# Autodesk Inventor assembly: WheelAssembly
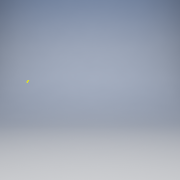
[picture p0: Inventor's stored thumbnail of the model, 180x180]
Saved by Autodesk Inventor 2016 (Build 200138000, 138)
## iProperties
Created: 2016-09-10
Part Number: WheelAssembly
Document SubType Name: Assembly
Designer: RoboticsUser
Author: RoboticsUser
## Documents named in this file (11)
- C:\Robotics\2016-17_CAD\WheelAssembly.iam
- C:\Robotics\CAD\2015-16\custom cad parts\am-2648_4inWheel8mmHub.ipt
- C:\Robotics\CAD\2015-16\COTSParts\Actobotics\545 parts\545556.ipt
- C:\Robotics\CAD\2015-16\COTSParts\Actobotics\615 parts\615102.ipt
- C:\Robotics\CAD\2015-16\COTSParts\Actobotics\634 parts\634080.ipt
- C:\Users\RoboticsUser\Desktop\2015-16 CAD\COTSParts\Actobotics\am-2964NeveRest.ipt
- C:\Users\RoboticsUser\Desktop\2015-16 CAD\COTSParts\Actobotics\615 parts\615114.ipt
- C:\Users\RoboticsUser\Desktop\2015-16 CAD\COTSParts\Tetrix\tetrix-motor-mounts-1.snapshot.1\Tetrex 2pc motor mount.ipt
- C:\Robotics\2016-17_CAD\DriveTrainPlate.iam
- C:\Robotics\CAD\2015-16\COTSParts\Actobotics\545 parts\545456.ipt
- C:\Robotics\CAD\2015-16\COTSParts\Bosch Extrusion\Bosch 20x20.ipt
## Components (26 placed, 10 different names)
1. am-2648_4inWheel8mmHub:2 — Insert:45, Insert:49
2. 545556:2 — Insert:48, Insert:51
3. 634080:1
4. 615102:3
5. 615102:4 — Insert:44
6. 634080:2 — Insert:41, Insert:47
7. am-2648_4inWheel8mmHub:3 — Insert:56, Insert:57
8. 545556:6 — Insert:52, Insert:55
9. 615102:5 — Insert:54, Insert:57
10. 634080:3 — Insert:40, Insert:46
11. am-2964NeveRest:2 — Insert:27, Insert:60
12. 545556:8 — Insert:61
13. 615114:2 — Insert:60, Insert:61
14. 615114:3 — Insert:58, Insert:59
15. 545556:9 — Insert:59
16. am-2964NeveRest:3 — Insert:28, Insert:58
17. Tetrex 2pc motor mount:1 — Insert:27, Insert:31, Insert:32, Insert:33
18. Tetrex 2pc motor mount:2 — Insert:28, Insert:34, Insert:35
19. DriveTrainPlate:1 [sub-assembly] — Insert:31, Insert:32, Insert:33, Insert:34, Insert:35, Insert:46, Insert:47, Mate:1, Flush:1, Flush:2
20. DriveTrainPlate:2 [sub-assembly] — Insert:40, Insert:41, Insert:51, Insert:52
21. 545556:10 — Insert:44, Insert:45
22. 545456:1 — Insert:49, Insert:48
23. 545456:2
24. 545456:3 — Insert:55, Insert:56
25. 545556:11 — Insert:54
26. Bosch 20x20:1 — Mate:1, Flush:1, Flush:2
## Relationships (28: Insert 25, Flush 2, Mate 1)
- Insert:27: am-2964NeveRest:2 ↔ Tetrex 2pc motor mount:1
- Insert:28: am-2964NeveRest:3 ↔ Tetrex 2pc motor mount:2
- Insert:31: Tetrex 2pc motor mount:1 ↔ DriveTrainPlate:1
- Insert:32: Tetrex 2pc motor mount:1 ↔ DriveTrainPlate:1
- Insert:33: Tetrex 2pc motor mount:1 ↔ DriveTrainPlate:1
- Insert:34: Tetrex 2pc motor mount:2 ↔ DriveTrainPlate:1
- Insert:35: Tetrex 2pc motor mount:2 ↔ DriveTrainPlate:1
- Insert:40: 634080:3 ↔ DriveTrainPlate:2
- Insert:41: 634080:2 ↔ DriveTrainPlate:2
- Insert:44: 615102:4 ↔ 545556:10
- Insert:45 (9.525 mm): am-2648_4inWheel8mmHub:2 ↔ 545556:10
- Insert:46 (2.3368 mm): 634080:3 ↔ DriveTrainPlate:1
- Insert:47 (2.3368 mm): 634080:2 ↔ DriveTrainPlate:1
- Insert:48: 545556:2 ↔ 545456:1
- Insert:49: am-2648_4inWheel8mmHub:2 ↔ 545456:1
- Insert:51 (9.525 mm): 545556:2 ↔ DriveTrainPlate:2
- Insert:52 (9.525 mm): 545556:6 ↔ DriveTrainPlate:2
- Insert:54: 615102:5 ↔ 545556:11
- Insert:55: 545556:6 ↔ 545456:3
- Insert:56: am-2648_4inWheel8mmHub:3 ↔ 545456:3
- Insert:57 (9.525 mm): am-2648_4inWheel8mmHub:3 ↔ 615102:5
- Insert:58 (16.637 mm): 615114:3 ↔ am-2964NeveRest:3
- Insert:59: 615114:3 ↔ 545556:9
- Insert:60 (16.637 mm): am-2964NeveRest:2 ↔ 615114:2
- Insert:61: 545556:8 ↔ 615114:2
- Mate:1: DriveTrainPlate:1 ↔ Bosch 20x20:1
- Flush:1: DriveTrainPlate:1 ↔ Bosch 20x20:1
- Flush:2: DriveTrainPlate:1 ↔ Bosch 20x20:1
